# Autodesk Inventor assembly: jorge's assembly
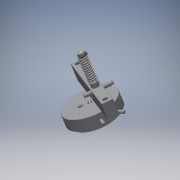
[picture p0: Inventor's stored thumbnail of the model, 180x180]
Saved by Autodesk Inventor 2017.3 (Build 213256000, 256)
## iProperties
Created: 2017-04-26
Part Number: jorge's assembly
Document SubType Name: Assembly
Designer: 167942
Author: 167942
## Documents named in this file (9)
- C:\Users\rbibb\Desktop\8.1\jorge's assembly.iam
- C:\Users\rbibb\Desktop\8.1\handle pivot pin.ipt
- C:\Users\rbibb\Desktop\8.1\upper die center support.ipt
- C:\Users\rbibb\Desktop\8.1\upper die pressure ring.ipt
- C:\Users\rbibb\Desktop\8.1\upper die center pin.ipt
- C:\Users\rbibb\Desktop\8.1\Large Snap Ring.ipt
- C:\Users\rbibb\Desktop\8.1\Upper Die Spring (1).ipt
- C:\Users\rbibb\Desktop\8.1\upper die outter ring.ipt
- C:\Users\rbibb\Desktop\8.1\upper die center.ipt
## Components (8 placed, 8 different names)
1. handle pivot pin:1 — Cylindrical:1
2. upper die center support:1 — Cylindrical:1, Rigid:1, Rotational:3
3. upper die pressure ring:1 — Rotational:3, Rotational:9, Rotational:10
4. upper die center pin:1 — Rigid:1, Rotational:7
5. Large Snap Ring:1 — Rotational:7, Rotational:8
6. Upper Die Spring (1):1 — Rotational:8
7. upper die outter ring:1 — Rotational:9
8. upper die center:1 — Rotational:10
## Relationships (7: RevoluteJoint 5, CylindricalJoint 1, WeldJoint 1)
- Cylindrical:1: handle pivot pin:1 ↔ upper die center support:1
- Rigid:1 [WeldJoint]: upper die center support:1 ↔ upper die center pin:1
- Rotational:3 [RevoluteJoint]: upper die center support:1 ↔ upper die pressure ring:1
- Rotational:7 [RevoluteJoint]: upper die center pin:1 ↔ Large Snap Ring:1
- Rotational:8 [RevoluteJoint]: Large Snap Ring:1 ↔ Upper Die Spring (1):1
- Rotational:9 [RevoluteJoint]: upper die pressure ring:1 ↔ upper die outter ring:1
- Rotational:10 [RevoluteJoint]: upper die pressure ring:1 ↔ upper die center:1
